# Autodesk Inventor assembly: MPPC
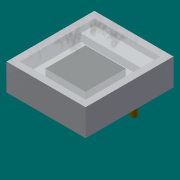
[picture p0: Inventor's stored thumbnail of the model, 180x180]
Saved by Autodesk Inventor 2016 (Build 200138000, 138)
## iProperties
Created: 2015-10-16
Part Number: MPPC
Document SubType Name: Assembly
Designer: Sawaiz
Author: Sawaiz
## Documents named in this file (3)
- C:\Users\Sawaiz\OneDrive\projects\mppcSensorInterface\cad\electronics\MPPC\MPPC.iam
- C:\Users\Sawaiz\OneDrive\projects\mppcSensorInterface\cad\electronics\MPPC\MPPC.ipt
- C:\Users\Sawaiz\OneDrive\projects\mppcSensorInterface\cad\electronics\MPPC\mppcLens.ipt
## Components (2 placed, 2 different names)
1. MPPC:1 — Flush:1, Flush:2
2. mppcLens:1 — Flush:1, Flush:2
## Relationships (2: Flush 2)
- Flush:1: MPPC:1 ↔ mppcLens:1
- Flush:2: MPPC:1 ↔ mppcLens:1
